# Autodesk Inventor assembly: wheel and axel bottom
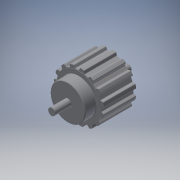
[picture p0: Inventor's stored thumbnail of the model, 180x180]
Saved by Autodesk Inventor 2016 (Build 200138000, 138)
## iProperties
Created: 2015-10-30
Part Number: wheel and axel bottom
Document SubType Name: Assembly
Designer: Delta
Author: Delta
## Documents named in this file (3)
- C:\Robotics\2015-16_CAD\custom cad parts\wheel and axel bottom.iam
- C:\Robotics\2015-16_CAD\custom cad parts\custom .25 in axel.ipt
- C:\Robotics\2015-16_CAD\custom cad parts\Pulley_no_side_15.ipt
## Components (2 placed, 2 different names)
1. custom .25 in axel:1 — Insert:1
2. Pulley_no_side_15:1 — Insert:1
## Relationships (1: Insert 1)
- Insert:1 (-14.925 mm): custom .25 in axel:1 ↔ Pulley_no_side_15:1
